# Autodesk Inventor assembly: Observatory
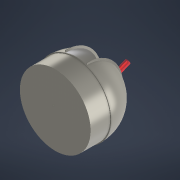
[picture p0: Inventor's stored thumbnail of the model, 180x180]
Saved by Autodesk Inventor 2022 (Build 260153000, 153)
## iProperties
Created: 2021-05-12
Part Number: Observatory
Document SubType Name: Assembly
Designer: Mick Veldhuis
Author: Mick Veldhuis
## Documents named in this file (15)
- C:\Users\Mick Veldhuis\Desktop\bsc-project\inventor\observatory\Observatory.iam
- C:\Users\Mick Veldhuis\Desktop\bsc-project\inventor\observatory\Dome\DomeFloor.ipt
- C:\Users\Mick Veldhuis\Desktop\bsc-project\inventor\observatory\Telescope\MountBase.ipt
- C:\Users\Mick Veldhuis\Desktop\bsc-project\inventor\observatory\Telescope\RaAxis.ipt
- C:\Users\Mick Veldhuis\Desktop\bsc-project\inventor\observatory\Telescope\Connectors\RaDecConnector.ipt
- C:\Users\Mick Veldhuis\Desktop\bsc-project\inventor\observatory\Telescope\DecAxis.ipt
- C:\Users\Mick Veldhuis\Desktop\bsc-project\inventor\observatory\Telescope\PrimaryMirror.ipt
- PrimaryMirror.ipt
- C:\Users\Mick Veldhuis\Desktop\bsc-project\inventor\observatory\Telescope\Connectors\TelescopeMountConnector.ipt
- C:\Users\Mick Veldhuis\Desktop\bsc-project\inventor\observatory\Telescope\GuiderWithFinder.ipt
- C:\Users\Mick Veldhuis\Desktop\bsc-project\inventor\observatory\Dome\DomeHemisphere.ipt
- C:\Users\Mick Veldhuis\Desktop\bsc-project\inventor\observatory\Telescope\Beams\Beam.ipt
- C:\Users\Mick Veldhuis\Desktop\bsc-project\inventor\observatory\Telescope\weights.ipt
- C:\Users\Mick Veldhuis\Desktop\bsc-project\inventor\observatory\Telescope\Beams\FinderBeam.ipt
- C:\Users\Mick Veldhuis\Desktop\bsc-project\inventor\observatory\Telescope\Beams\GuiderBeam.ipt
## Components (15 placed, 13 different names)
1. DomeFloor:1 — Insert:1, Insert:2, AzAxisRotation
2. DomeHemisphere:1 — AzAxisRotation
3. RaAxis:1 — RaAxisRotation, Insert:3, Insert:4
4. DecAxis:1 — DecAxisRotation, Insert:9, Insert:10, Insert:14, Insert:15
5. MountBase:1 — Insert:1, Insert:2, RaAxisRotation
6. RaDecConnector:1 — Insert:3, Insert:4, DecAxisRotation
7. PrimaryMirror:1 — Insert:5, Insert:6, Insert:7, Insert:8, Insert:11, Insert:12, Insert:13
8. TelescopeMountConnector:1 — Insert:5, Insert:6, Insert:10
9. TelescopeMountConnector:2 — Insert:7, Insert:8, Insert:9
10. GuiderWithFinder:1 — Insert:11, Insert:12, Insert:16, Insert:17
11. weights:1 — Insert:14
12. weights:2 — Insert:15
13. Beam:1 — Insert:13
14. FinderBeam:1 — Insert:17
15. GuiderBeam:1 — Insert:16
## Relationships (20: Insert 17, RevoluteJoint 2, CylindricalJoint 1)
- Insert:1: DomeFloor:1 ↔ MountBase:1
- Insert:2: DomeFloor:1 ↔ MountBase:1
- RaAxisRotation [RevoluteJoint]: RaAxis:1 ↔ MountBase:1
- Insert:3: RaAxis:1 ↔ RaDecConnector:1
- Insert:4: RaAxis:1 ↔ RaDecConnector:1
- DecAxisRotation [RevoluteJoint]: DecAxis:1 ↔ RaDecConnector:1
- Insert:5: PrimaryMirror:1 ↔ TelescopeMountConnector:1
- Insert:6: PrimaryMirror:1 ↔ TelescopeMountConnector:1
- Insert:7: PrimaryMirror:1 ↔ TelescopeMountConnector:2
- Insert:8: PrimaryMirror:1 ↔ TelescopeMountConnector:2
- Insert:9: DecAxis:1 ↔ TelescopeMountConnector:2
- Insert:10: DecAxis:1 ↔ TelescopeMountConnector:1
- Insert:11: PrimaryMirror:1 ↔ GuiderWithFinder:1
- Insert:12: PrimaryMirror:1 ↔ GuiderWithFinder:1
- Insert:13: PrimaryMirror:1 ↔ Beam:1
- Insert:14 (180 mm): DecAxis:1 ↔ weights:1
- Insert:15 (90 mm): DecAxis:1 ↔ weights:2
- Insert:16: GuiderWithFinder:1 ↔ GuiderBeam:1
- Insert:17 (-50 mm): GuiderWithFinder:1 ↔ FinderBeam:1
- AzAxisRotation [CylindricalJoint]: DomeFloor:1 ↔ DomeHemisphere:1
